# Autodesk Inventor assembly: ASY NDM 11.036 укосина
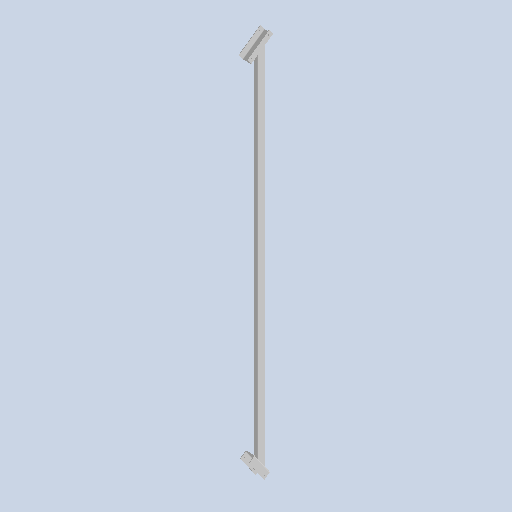
[picture p0: Inventor's stored thumbnail of the model, 512x512]
Saved by Autodesk Inventor 2025 (Build 290162010, 162A)
## iProperties
Created: 2024-08-18
Part Number: ASY NDM 11.036 укосина
Document SubType Name: Assembly
Designer: admin
Author: admin
## Documents named in this file (3)
- C:\Users\admin\YandexDisk-badmisterfox\домашниий пк\Inventor\Nadyim\CAD\Перегородка\ASY NDM 11.036 укосина.iam
- C:\Users\admin\YandexDisk-badmisterfox\домашниий пк\Inventor\Nadyim\CAD\Перегородка\NDM 11.033 перегородка укосина.ipt
- C:\Users\admin\YandexDisk-badmisterfox\домашниий пк\Inventor\Nadyim\CAD\кронштейн\NDM 11.027 кронштейн 27.ipt
## Components (3 placed, 2 different names)
1. NDM 11.033 перегородка укосина:1 — Rigid:3, Rigid:4
2. NDM 11.027 кронштейн 27:1 — Rigid:3
3. NDM 11.027 кронштейн 27:2 — Rigid:4
## Relationships (2: WeldJoint 2)
- Rigid:3 [WeldJoint]: NDM 11.033 перегородка укосина:1 ↔ NDM 11.027 кронштейн 27:1
- Rigid:4 [WeldJoint]: NDM 11.033 перегородка укосина:1 ↔ NDM 11.027 кронштейн 27:2
